# Autodesk Inventor assembly: SPE1V1 Estructura
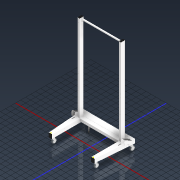
[picture p0: Inventor's stored thumbnail of the model, 180x180]
Saved by Autodesk Inventor 2021.2 (Build 252289000, 289)
## iProperties
Created: 2026-06-02
Part Number: SPE1V1 Estructura
Document SubType Name: Assembly
Designer: nelso
Mass: 32774.5 g
Surface Area: 45303.3 cm^2
Volume: 6303.93 cm^3
Density: 5.19906 g/cm^3
Author: nelso
## Documents named in this file (21)
- C:\Users\Tecnica\OneDrive\Documentos\Mecanica\Soporte-Paciente-Espinografia\Workspace\SPE1V1 Estructura.iam
- C:\Users\Tecnica\OneDrive\Documentos\Mecanica\Soporte-Paciente-Espinografia\Workspace\SP28V1 Tapacanto Delantero.ipt
- C:\Users\Tecnica\OneDrive\Documentos\Mecanica\Soporte-Paciente-Espinografia\Workspace\SP27V1 Tapacanto Superior.ipt
- C:\Users\Tecnica\OneDrive\Documentos\Mecanica\Soporte-Paciente-Espinografia\Workspace\RFPLUS8PO300.ipt
- C:\Users\Tecnica\OneDrive\Documentos\Mecanica\Soporte-Paciente-Espinografia\Workspace\SP26V1 Varilla Pedal.ipt
- C:\Users\Tecnica\OneDrive\Documentos\Mecanica\Soporte-Paciente-Espinografia\Workspace\SP23V1 Pedal Izquierdo.ipt
- C:\Users\Tecnica\OneDrive\Documentos\Mecanica\Soporte-Paciente-Espinografia\Workspace\SPE9V1 Freno.iam
- C:\Users\Tecnica\OneDrive\Documentos\Mecanica\Soporte-Paciente-Espinografia\Workspace\G3-100-PPP-RU.ipt
- C:\Users\Tecnica\OneDrive\Documentos\Mecanica\Soporte-Paciente-Espinografia\Workspace\DIN 555A10C.ipt
- C:\Users\Tecnica\OneDrive\Documentos\Mecanica\Soporte-Paciente-Espinografia\Workspace\DIN125-A8,4C.ipt
- C:\Users\Tecnica\OneDrive\Documentos\Mecanica\Soporte-Paciente-Espinografia\Workspace\DIN933M8X1.25L20C.ipt
- C:\Users\Tecnica\OneDrive\Documentos\Mecanica\Soporte-Paciente-Espinografia\Workspace\SP25V1 Seguro Pedales.ipt
- C:\Users\Tecnica\OneDrive\Documentos\Mecanica\Soporte-Paciente-Espinografia\Workspace\ISO7380M6X1L12I.ipt
- C:\Users\Tecnica\OneDrive\Documentos\Mecanica\Soporte-Paciente-Espinografia\Workspace\ISO7380M4X0.8L12I.ipt
- C:\Users\Tecnica\OneDrive\Documentos\Mecanica\Soporte-Paciente-Espinografia\Workspace\DIN555-5M4X0.8I.ipt
- C:\Users\Tecnica\OneDrive\Documentos\Mecanica\Soporte-Paciente-Espinografia\Workspace\SP24V1 Goma Pedales.ipt
- C:\Users\Tecnica\OneDrive\Documentos\Mecanica\Soporte-Paciente-Espinografia\Workspace\SPE8V1 Estructura (soldadura).iam
- C:\Users\Tecnica\OneDrive\Documentos\Mecanica\Soporte-Paciente-Espinografia\Workspace\SPE11V1 Baranda Superior (soldadura).iam
- C:\Users\Tecnica\OneDrive\Documentos\Mecanica\Soporte-Paciente-Espinografia\Workspace\DIN125-A6.4.ipt
- C:\Users\Tecnica\OneDrive\Documentos\Mecanica\Soporte-Paciente-Espinografia\Workspace\DIN125-A4.3.ipt
- C:\Users\Tecnica\OneDrive\Documentos\Mecanica\Soporte-Paciente-Espinografia\Workspace\SP22V1 Pedal Derecho.ipt
## Components (67 placed, 20 different names)
1. SPE8V1 Estructura (soldadura):1 [sub-assembly]
2. SPE9V1 Freno:1 [sub-assembly] — Flush:103, Mate:117, Mate:118, Mate:119
3. SPE9V1 Freno:2 [sub-assembly] — Flush:103, Mate:133, Mate:134
4. SPE11V1 Baranda Superior (soldadura):1 [sub-assembly]
5. SP22V1 Pedal Derecho:1 — Mate:302, Mate:303, Mate:304, Mate:305, Mate:306, Mate:307, Mate:308, Mate:309, Mate:310, Mate:311
6. SP23V1 Pedal Izquierdo:1 — Mate:297, Mate:298, Mate:299, Mate:327, Mate:328, Mate:329, Flush:151, Mate:330, Mate:333
7. SP24V1 Goma Pedales:1 — Mate:302, Mate:303, Mate:304
8. SP24V1 Goma Pedales:2 — Mate:297, Mate:298, Mate:299
9. SP25V1 Seguro Pedales:1 — Mate:315, Mate:316, Mate:317, Mate:330, Mate:331, Mate:332
10. SP25V1 Seguro Pedales:2 — Mate:272, Mate:273, Mate:309, Mate:312
11. SP26V1 Varilla Pedal:1 — Mate:117, Mate:118, Mate:119, Mate:133, Mate:134, Mate:258, Mate:305, Mate:306, Mate:312, Mate:325, Mate:328, Mate:329, Flush:151
12. SP27V1 Tapacanto Superior:1
13. SP27V1 Tapacanto Superior:2
14. SP28V1 Tapacanto Delantero:1
15. SP28V1 Tapacanto Delantero:2
16. RFPLUS8PO300:1
17. RFPLUS8PO300:2
18. RFPLUS8PO300:3
19. RFPLUS8PO300:4
20. RFPLUS8PO300:5
21. RFPLUS8PO300:6
22. RFPLUS8PO300:17
23. RFPLUS8PO300:18
24. RFPLUS8PO300:19
25. RFPLUS8PO300:20
26. RFPLUS8PO300:21
27. RFPLUS8PO300:22
28. RFPLUS8PO300:23 — Mate:223
29. RFPLUS8PO300:24 — Mate:224
30. RFPLUS8PO300:25
31. RFPLUS8PO300:26
32. G3-100-PPP-RU:1
33. G3-100-PPP-RU:2
34. G3-100-PPP-RU:3
35. G3-100-PPP-RU:4
36. DIN 555A10C:1
37. DIN 555A10C:2
38. DIN 555A10C:3
39. DIN 555A10C:4
40. DIN125-A8,4C:1 — Mate:214, Mate:215
41. DIN125-A8,4C:2 — Mate:216, Mate:217
42. DIN125-A8,4C:3
43. DIN125-A8,4C:4
44. DIN933M8X1.25L20C:1 — Mate:214, Mate:215, Mate:224
45. DIN933M8X1.25L20C:2 — Mate:216, Mate:217, Mate:223
46. DIN933M8X1.25L20C:3
47. DIN933M8X1.25L20C:4
48. ISO7380M6X1L12I:1 — Mate:258
49. ISO7380M6X1L12I:2 — Mate:323, Mate:324, Mate:325, Mate:332
50. DIN125-A6.4:1
51. DIN125-A6.4:2 — Mate:323, Mate:324, Mate:331
52. ISO7380M4X0.8L12I:1 — Mate:282, Mate:317, Mate:320
53. ISO7380M4X0.8L12I:2 — Mate:284, Mate:313, Mate:314, Mate:315, Mate:321, Mate:333
54. ISO7380M4X0.8L12I:3 — Mate:273, Mate:288, Mate:308
55. ISO7380M4X0.8L12I:4 — Mate:272, Mate:289, Mate:307
56. DIN125-A4.3:1 — Mate:313, Mate:314, Mate:316
57. DIN125-A4.3:2
58. DIN125-A4.3:3
59. DIN125-A4.3:4
60. DIN125-A4.3:5 — Mate:321, Mate:322
61. DIN125-A4.3:6 — Mate:320, Mate:326, Mate:327
62. DIN125-A4.3:7 — Mate:311
63. DIN125-A4.3:8 — Mate:310
64. DIN555-5M4X0.8I:1 — Mate:282, Mate:326
65. DIN555-5M4X0.8I:2 — Mate:284, Mate:322
66. DIN555-5M4X0.8I:3 — Mate:289
67. DIN555-5M4X0.8I:4 — Mate:288
## Relationships (163: Mate 130, Flush 33)
- [Mate]: SPE8V1 Estructura (soldadura):1 ↔ SP27V1 Tapacanto Superior:1
- [Flush]: SPE8V1 Estructura (soldadura):1 ↔ SP27V1 Tapacanto Superior:1
- [Mate]: SPE8V1 Estructura (soldadura):1 ↔ SP27V1 Tapacanto Superior:1
- [Flush]: SPE8V1 Estructura (soldadura):1 ↔ RFPLUS8PO300:2
- [Flush]: SPE8V1 Estructura (soldadura):1 ↔ RFPLUS8PO300:3
- [Flush]: SPE8V1 Estructura (soldadura):1 ↔ RFPLUS8PO300:4
- [Flush]: SPE8V1 Estructura (soldadura):1 ↔ RFPLUS8PO300:5
- [Flush]: SPE8V1 Estructura (soldadura):1 ↔ RFPLUS8PO300:6
- [Mate]: SPE8V1 Estructura (soldadura):1 ↔ RFPLUS8PO300:5
- [Mate]: SPE8V1 Estructura (soldadura):1 ↔ RFPLUS8PO300:6
- [Mate]: SPE8V1 Estructura (soldadura):1 ↔ RFPLUS8PO300:4
- [Mate]: SPE8V1 Estructura (soldadura):1 ↔ RFPLUS8PO300:3
- [Mate]: SPE8V1 Estructura (soldadura):1 ↔ RFPLUS8PO300:2
- [Mate]: SPE8V1 Estructura (soldadura):1 ↔ RFPLUS8PO300:1
- [Flush]: SPE8V1 Estructura (soldadura):1 ↔ RFPLUS8PO300:1
- [Mate]: SPE8V1 Estructura (soldadura):1 ↔ SPE9V1 Freno:1
- [Mate]: SPE8V1 Estructura (soldadura):1 ↔ SPE9V1 Freno:2
- Flush:103: SPE9V1 Freno:1 ↔ SPE9V1 Freno:2
- Mate:117: SPE9V1 Freno:1 ↔ SP26V1 Varilla Pedal:1
- Mate:118: SPE9V1 Freno:1 ↔ SP26V1 Varilla Pedal:1
- Mate:119: SPE9V1 Freno:1 ↔ SP26V1 Varilla Pedal:1
- [Mate]: SPE8V1 Estructura (soldadura):1 ↔ SPE9V1 Freno:1
- [Mate]: SPE8V1 Estructura (soldadura):1 ↔ SP26V1 Varilla Pedal:1
- [Mate] (100 mm): SPE8V1 Estructura (soldadura):1 ↔ SPE9V1 Freno:2
- [Mate] (100 mm): SPE8V1 Estructura (soldadura):1 ↔ SPE9V1 Freno:1
- Mate:133: SPE9V1 Freno:2 ↔ SP26V1 Varilla Pedal:1
- Mate:134: SPE9V1 Freno:2 ↔ SP26V1 Varilla Pedal:1
- [Flush]: SPE8V1 Estructura (soldadura):1 ↔ SP27V1 Tapacanto Superior:2
- [Mate]: SPE8V1 Estructura (soldadura):1 ↔ SP27V1 Tapacanto Superior:2
- [Mate]: SPE8V1 Estructura (soldadura):1 ↔ G3-100-PPP-RU:4
- [Mate]: SPE8V1 Estructura (soldadura):1 ↔ SP27V1 Tapacanto Superior:2
- [Mate]: SPE8V1 Estructura (soldadura):1 ↔ RFPLUS8PO300:21
- [Mate]: SPE8V1 Estructura (soldadura):1 ↔ RFPLUS8PO300:22
- [Mate]: SPE8V1 Estructura (soldadura):1 ↔ RFPLUS8PO300:20
- [Mate]: SPE8V1 Estructura (soldadura):1 ↔ RFPLUS8PO300:19
- [Mate]: SPE8V1 Estructura (soldadura):1 ↔ RFPLUS8PO300:18
- [Mate]: SPE8V1 Estructura (soldadura):1 ↔ RFPLUS8PO300:17
- [Flush]: SPE8V1 Estructura (soldadura):1 ↔ RFPLUS8PO300:17
- [Flush]: SPE8V1 Estructura (soldadura):1 ↔ RFPLUS8PO300:18
- [Flush]: SPE8V1 Estructura (soldadura):1 ↔ RFPLUS8PO300:19
- [Flush]: SPE8V1 Estructura (soldadura):1 ↔ RFPLUS8PO300:20
- [Flush]: SPE8V1 Estructura (soldadura):1 ↔ RFPLUS8PO300:21
- [Flush]: SPE8V1 Estructura (soldadura):1 ↔ RFPLUS8PO300:22
- [Mate]: SPE8V1 Estructura (soldadura):1 ↔ DIN 555A10C:3
- [Mate]: SPE8V1 Estructura (soldadura):1 ↔ DIN 555A10C:4
- [Mate]: SPE8V1 Estructura (soldadura):1 ↔ DIN 555A10C:2
- [Mate]: SPE8V1 Estructura (soldadura):1 ↔ DIN 555A10C:1
- [Mate]: SPE8V1 Estructura (soldadura):1 ↔ DIN 555A10C:1
- [Mate]: SPE8V1 Estructura (soldadura):1 ↔ DIN 555A10C:2
- [Mate]: SPE8V1 Estructura (soldadura):1 ↔ DIN 555A10C:3
- [Mate]: SPE8V1 Estructura (soldadura):1 ↔ DIN 555A10C:4
- [Flush]: SPE8V1 Estructura (soldadura):1 ↔ SP26V1 Varilla Pedal:1
- [Flush] (7.5 mm): SPE8V1 Estructura (soldadura):1
- [Flush] (7.5 mm): SPE8V1 Estructura (soldadura):1
- [Mate]: SPE8V1 Estructura (soldadura):1 ↔ G3-100-PPP-RU:3
- [Mate]: SPE8V1 Estructura (soldadura):1 ↔ G3-100-PPP-RU:3
- [Flush]: SPE8V1 Estructura (soldadura):1 ↔ G3-100-PPP-RU:3
- [Mate]: SPE8V1 Estructura (soldadura):1 ↔ G3-100-PPP-RU:2
- [Mate]: SPE8V1 Estructura (soldadura):1 ↔ G3-100-PPP-RU:2
- [Flush]: SPE8V1 Estructura (soldadura):1 ↔ G3-100-PPP-RU:2
- [Mate]: SPE8V1 Estructura (soldadura):1 ↔ G3-100-PPP-RU:4
- [Flush]: SPE8V1 Estructura (soldadura):1 ↔ G3-100-PPP-RU:4
- [Mate]: SPE8V1 Estructura (soldadura):1 ↔ G3-100-PPP-RU:1
- [Flush]: SPE8V1 Estructura (soldadura):1 ↔ G3-100-PPP-RU:1
- [Mate]: SPE8V1 Estructura (soldadura):1 ↔ G3-100-PPP-RU:1
- [Mate]: SPE8V1 Estructura (soldadura):1 ↔ SP28V1 Tapacanto Delantero:1
- [Flush]: SPE8V1 Estructura (soldadura):1
- [Mate]: SPE8V1 Estructura (soldadura):1
- [Flush]: SPE8V1 Estructura (soldadura):1
- [Mate] (380 mm): SPE8V1 Estructura (soldadura):1
- [Flush]: SPE8V1 Estructura (soldadura):1 ↔ SP28V1 Tapacanto Delantero:2
- [Flush]: SPE8V1 Estructura (soldadura):1 ↔ SP28V1 Tapacanto Delantero:2
- [Mate]: SPE8V1 Estructura (soldadura):1 ↔ SP28V1 Tapacanto Delantero:2
- [Flush]: SPE8V1 Estructura (soldadura):1 ↔ SP28V1 Tapacanto Delantero:1
- [Flush]: SPE8V1 Estructura (soldadura):1 ↔ SP28V1 Tapacanto Delantero:1
- Mate:214: DIN125-A8,4C:1 ↔ DIN933M8X1.25L20C:1
- Mate:215: DIN125-A8,4C:1 ↔ DIN933M8X1.25L20C:1
- Mate:216: DIN125-A8,4C:2 ↔ DIN933M8X1.25L20C:2
- Mate:217: DIN125-A8,4C:2 ↔ DIN933M8X1.25L20C:2
- [Mate]: SPE11V1 Baranda Superior (soldadura):1 ↔ DIN125-A8,4C:2
- [Mate]: SPE11V1 Baranda Superior (soldadura):1 ↔ DIN125-A8,4C:1
- [Mate]: SPE11V1 Baranda Superior (soldadura):1 ↔ DIN933M8X1.25L20C:1
- [Mate]: SPE11V1 Baranda Superior (soldadura):1 ↔ DIN933M8X1.25L20C:2
- [Mate]: SPE8V1 Estructura (soldadura):1 ↔ SPE11V1 Baranda Superior (soldadura):1
- [Flush]: SPE8V1 Estructura (soldadura):1 ↔ RFPLUS8PO300:24
- [Flush]: SPE8V1 Estructura (soldadura):1 ↔ RFPLUS8PO300:23
- Mate:223: RFPLUS8PO300:23 ↔ DIN933M8X1.25L20C:2
- Mate:224: RFPLUS8PO300:24 ↔ DIN933M8X1.25L20C:1
- [Mate]: DIN125-A8,4C:3 ↔ DIN933M8X1.25L20C:3
- [Mate]: DIN125-A8,4C:3 ↔ DIN933M8X1.25L20C:3
- [Mate]: DIN125-A8,4C:4 ↔ DIN933M8X1.25L20C:4
- [Mate]: DIN125-A8,4C:4 ↔ DIN933M8X1.25L20C:4
- [Mate]: SPE11V1 Baranda Superior (soldadura):1 ↔ DIN125-A8,4C:4
- [Mate]: SPE11V1 Baranda Superior (soldadura):1 ↔ DIN125-A8,4C:3
- [Mate]: SPE11V1 Baranda Superior (soldadura):1 ↔ DIN933M8X1.25L20C:3
- [Mate]: SPE11V1 Baranda Superior (soldadura):1 ↔ DIN933M8X1.25L20C:4
- [Mate]: RFPLUS8PO300:25 ↔ DIN933M8X1.25L20C:4
- [Mate]: RFPLUS8PO300:26 ↔ DIN933M8X1.25L20C:3
- [Mate]: SPE8V1 Estructura (soldadura):1 ↔ SPE11V1 Baranda Superior (soldadura):1
- [Flush]: SPE8V1 Estructura (soldadura):1 ↔ RFPLUS8PO300:26
- [Flush]: SPE8V1 Estructura (soldadura):1 ↔ RFPLUS8PO300:25
- [Mate]: SPE8V1 Estructura (soldadura):1 ↔ DIN933M8X1.25L20C:1
- [Mate]: SPE8V1 Estructura (soldadura):1 ↔ DIN933M8X1.25L20C:2
- [Mate]: SPE8V1 Estructura (soldadura):1 ↔ DIN933M8X1.25L20C:3
- [Mate]: SPE8V1 Estructura (soldadura):1 ↔ DIN933M8X1.25L20C:4
- [Mate]: SPE11V1 Baranda Superior (soldadura):1
- [Mate]: ISO7380M6X1L12I:1 ↔ DIN125-A6.4:1
- [Mate]: ISO7380M6X1L12I:1 ↔ DIN125-A6.4:1
- Mate:258: SP26V1 Varilla Pedal:1 ↔ ISO7380M6X1L12I:1
- [Mate]: SP25V1 Seguro Pedales:2 ↔ DIN125-A6.4:1
- [Mate]: ISO7380M4X0.8L12I:1 ↔ DIN125-A4.3:2
- [Mate]: ISO7380M4X0.8L12I:1 ↔ DIN125-A4.3:2
- [Mate]: ISO7380M4X0.8L12I:3 ↔ DIN125-A4.3:4
- [Mate]: ISO7380M4X0.8L12I:3 ↔ DIN125-A4.3:4
- [Mate]: ISO7380M4X0.8L12I:4 ↔ DIN125-A4.3:3
- [Mate]: ISO7380M4X0.8L12I:4 ↔ DIN125-A4.3:3
- [Mate]: SP25V1 Seguro Pedales:2 ↔ DIN125-A4.3:3
- [Mate]: SP25V1 Seguro Pedales:2 ↔ DIN125-A4.3:4
- Mate:272: SP25V1 Seguro Pedales:2 ↔ ISO7380M4X0.8L12I:4
- Mate:273: SP25V1 Seguro Pedales:2 ↔ ISO7380M4X0.8L12I:3
- [Mate]: SP25V1 Seguro Pedales:1 ↔ DIN125-A4.3:2
- [Mate]: ISO7380M4X0.8L12I:4 ↔ DIN125-A4.3:7
- [Mate]: ISO7380M4X0.8L12I:3 ↔ DIN125-A4.3:8
- Mate:282: ISO7380M4X0.8L12I:1 ↔ DIN555-5M4X0.8I:1
- Mate:284: ISO7380M4X0.8L12I:2 ↔ DIN555-5M4X0.8I:2
- Mate:288: ISO7380M4X0.8L12I:3 ↔ DIN555-5M4X0.8I:4
- Mate:289: ISO7380M4X0.8L12I:4 ↔ DIN555-5M4X0.8I:3
- [Mate]: DIN125-A4.3:7 ↔ DIN555-5M4X0.8I:3
- [Mate]: DIN125-A4.3:8 ↔ DIN555-5M4X0.8I:4
- Mate:297: SP23V1 Pedal Izquierdo:1 ↔ SP24V1 Goma Pedales:2
- Mate:298: SP23V1 Pedal Izquierdo:1 ↔ SP24V1 Goma Pedales:2
- Mate:299: SP23V1 Pedal Izquierdo:1 ↔ SP24V1 Goma Pedales:2
- Mate:302: SP22V1 Pedal Derecho:1 ↔ SP24V1 Goma Pedales:1
- Mate:303: SP22V1 Pedal Derecho:1 ↔ SP24V1 Goma Pedales:1
- Mate:304: SP22V1 Pedal Derecho:1 ↔ SP24V1 Goma Pedales:1
- Mate:305: SP22V1 Pedal Derecho:1 ↔ SP26V1 Varilla Pedal:1
- Mate:306: SP22V1 Pedal Derecho:1 ↔ SP26V1 Varilla Pedal:1
- Mate:307: SP22V1 Pedal Derecho:1 ↔ ISO7380M4X0.8L12I:4
- Mate:308: SP22V1 Pedal Derecho:1 ↔ ISO7380M4X0.8L12I:3
- Mate:309: SP22V1 Pedal Derecho:1 ↔ SP25V1 Seguro Pedales:2
- Mate:310: SP22V1 Pedal Derecho:1 ↔ DIN125-A4.3:8
- Mate:311: SP22V1 Pedal Derecho:1 ↔ DIN125-A4.3:7
- Mate:312: SP25V1 Seguro Pedales:2 ↔ SP26V1 Varilla Pedal:1
- Mate:313: ISO7380M4X0.8L12I:2 ↔ DIN125-A4.3:1
- Mate:314: ISO7380M4X0.8L12I:2 ↔ DIN125-A4.3:1
- Mate:315: SP25V1 Seguro Pedales:1 ↔ ISO7380M4X0.8L12I:2
- Mate:316: SP25V1 Seguro Pedales:1 ↔ DIN125-A4.3:1
- Mate:317: SP25V1 Seguro Pedales:1 ↔ ISO7380M4X0.8L12I:1
- Mate:320: ISO7380M4X0.8L12I:1 ↔ DIN125-A4.3:6
- Mate:321: ISO7380M4X0.8L12I:2 ↔ DIN125-A4.3:5
- Mate:322: DIN125-A4.3:5 ↔ DIN555-5M4X0.8I:2
- Mate:323: ISO7380M6X1L12I:2 ↔ DIN125-A6.4:2
- Mate:324: ISO7380M6X1L12I:2 ↔ DIN125-A6.4:2
- Mate:325: SP26V1 Varilla Pedal:1 ↔ ISO7380M6X1L12I:2
- Mate:326: DIN125-A4.3:6 ↔ DIN555-5M4X0.8I:1
- Mate:327: SP23V1 Pedal Izquierdo:1 ↔ DIN125-A4.3:6
- Mate:328: SP23V1 Pedal Izquierdo:1 ↔ SP26V1 Varilla Pedal:1
- Mate:329: SP23V1 Pedal Izquierdo:1 ↔ SP26V1 Varilla Pedal:1
- Flush:151: SP23V1 Pedal Izquierdo:1 ↔ SP26V1 Varilla Pedal:1
- Mate:330: SP23V1 Pedal Izquierdo:1 ↔ SP25V1 Seguro Pedales:1
- Mate:331: SP25V1 Seguro Pedales:1 ↔ DIN125-A6.4:2
- Mate:332: SP25V1 Seguro Pedales:1 ↔ ISO7380M6X1L12I:2
- Mate:333: SP23V1 Pedal Izquierdo:1 ↔ ISO7380M4X0.8L12I:2
## Named parameters: d314_d103 = 0 mm, d315_d104 = 0 mm, d464_d462 = 0 mm, d465_d463 = 0 mm, d466_d449 = 0 mm, d467_d450 = 0 mm, d468_d451 = 0 mm, d469_d452 = 0 mm, d470_d453 = 0 mm, d471_d454 = 0 mm, d472_d455 = 0 mm, d473_d456 = 0 mm
